# Autodesk Inventor assembly: 3-clamp
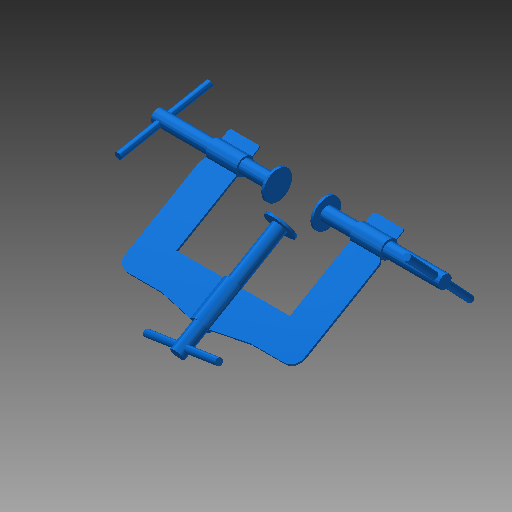
[picture p0: Inventor's stored thumbnail of the model, 512x512]
Saved by Autodesk Inventor 2018 (Build 220112000, 112)
## iProperties
Created: 2018-06-15
Part Number: 3-clamp
Material: 一般
Document SubType Name: Assembly
Designer: KITformula
Author: KITformula
## Documents named in this file (3)
- Z:\各班フォルダ\2018\ボディ\エアロ\Aero\KS-15\コスト用CAD\その他\3-Clamp.iam
- Z:\各班フォルダ\2018\ボディ\エアロ\Aero\KS-15\コスト用CAD\その他\3-clamp body.ipt
- Z:\各班フォルダ\2018\ボディ\エアロ\Aero\KS-15\コスト用CAD\その他\3-clamp shaft.ipt
## Components (4 placed, 4 different names)
1. 3-clamp body.1 — メイト:1, メイト:2, メイト:3
2. 3-clamp shaft.1 — メイト:1
3. 3-clamp shaft.2 — メイト:3
4. 3-clamp shaft.3 — メイト:2
## Relationships (3: Mate 3)
- メイト:1 [Mate]: 3-clamp body.1 ↔ 3-clamp shaft.1
- メイト:2 [Mate]: 3-clamp body.1 ↔ 3-clamp shaft.3
- メイト:3 [Mate]: 3-clamp body.1 ↔ 3-clamp shaft.2
